# Autodesk Inventor assembly: Mounted Pump
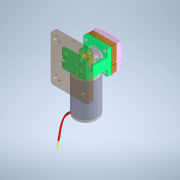
[picture p0: Inventor's stored thumbnail of the model, 180x180]
Saved by Autodesk Inventor 2021 (Build 250183000, 183)
## iProperties
Created: 2020-07-16
Part Number: Mounted Pump
Document SubType Name: Assembly
Designer: jgray
Author: jgray
## Documents named in this file (3)
- M:\Printed Electronics\Gas Sensors\Prototypes\Prototype II -Cartridge Reader V3\Mounted Pump.iam
- M:\Printed Electronics\Gas Sensors\Prototypes\Prototype II -Cartridge Reader V3\Pump GD 20020307-1820020307-18_20160204_bschn.ipt
- M:\Printed Electronics\Gas Sensors\Prototypes\Prototype II -Cartridge Reader V3\Pump Mounting Plate.ipt
## Components (2 placed, 2 different names)
1. Pump GD 20020307-1820020307-18_20160204_bschn:1 — Mate:1, Mate:2, Mate:3
2. Pump Mounting Plate:1 — Mate:1, Mate:2, Mate:3
## Relationships (3: Mate 3)
- Mate:1: Pump GD 20020307-1820020307-18_20160204_bschn:1 ↔ Pump Mounting Plate:1
- Mate:2: Pump GD 20020307-1820020307-18_20160204_bschn:1 ↔ Pump Mounting Plate:1
- Mate:3: Pump GD 20020307-1820020307-18_20160204_bschn:1 ↔ Pump Mounting Plate:1
